# Autodesk Inventor assembly: Inlet 3D print part
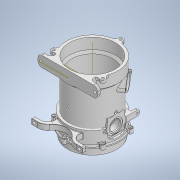
[picture p0: Inventor's stored thumbnail of the model, 180x180]
Saved by Autodesk Inventor 2020 (Build 240168000, 168)
## iProperties
Created: 2020-04-10
Part Number: Inlet 3D print part
Document SubType Name: Assembly
Designer: angusaitken
Author: angusaitken
## Documents named in this file (3)
- \\Mac\Home\Desktop\3D\Breeze thing\Breeze V2\Inlet subassembly stuff - Angus\Inlet 3D print part.iam
- \\Mac\Home\Desktop\3D\Breeze thing\Breeze V2\Inlet subassembly stuff - Angus\Inlet housing.ipt
- \\Mac\Home\Desktop\3D\Breeze thing\Breeze V2\Impeller Assembly\BRZ-P203.ipt
## Components (2 placed, 2 different names)
1. Inlet housing:1 — Mate:1, Flush:1, Angle:1
2. BRZ-P203:1 — Mate:1, Flush:1, Angle:1
## Relationships (3: Mate 1, Flush 1, Angle 1)
- Mate:1: Inlet housing:1 ↔ BRZ-P203:1
- Flush:1: Inlet housing:1 ↔ BRZ-P203:1
- Angle:1 (0 deg): Inlet housing:1 ↔ BRZ-P203:1
